# Autodesk Inventor assembly: Сборка2
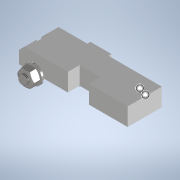
[picture p0: Inventor's stored thumbnail of the model, 180x180]
Saved by Autodesk Inventor 2022 (Build 260153000, 153)
## iProperties
Created: 2024-04-28
Part Number: Сборка2
Document SubType Name: Assembly
Designer: Pavel
Author: Pavel
## Documents named in this file (9)
- D:\BSUIR\КМЭКЭС\Сборка2.iam
- D:\BSUIR\КМЭКЭС\Исходники\Разрез\Деталь.ipt
- C:\Users\Pavel\Documents\Inventor\Content Center Files\R2022\ru-RU\Stud GOST 22032-76\Шпилька M10-6g×30 ГОСТ 22032-76.ipt
- C:\Users\Pavel\Documents\Inventor\Content Center Files\R2022\ru-RU\Washer 1 GOST 6402-78\Шайба 10Н ГОСТ 6402-78.ipt
- C:\Users\Pavel\Documents\Inventor\Content Center Files\R2022\ru-RU\GOST 5915-70\Гайка M10-6H ГОСТ 5915-70(1).ipt
- C:\Users\Pavel\Documents\Inventor\Content Center Files\R2022\ru-RU\Screw B GOST 17473-80\Винт B.M8-6gx25 ГОСТ 17473-80.ipt
- C:\Users\Pavel\Documents\Inventor\Content Center Files\R2022\ru-RU\Bolt GOST 7798-78\Болт M12-6g×60 ГОСТ 7798-70.ipt
- C:\Users\Pavel\Documents\Inventor\Content Center Files\R2022\ru-RU\GOST 11371-78  A\Шайба 12 ГОСТ 11371-78.ipt
- C:\Users\Pavel\Documents\Inventor\Content Center Files\R2022\ru-RU\GOST 5915-70\Гайка M12-6H ГОСТ 5915-70(1).ipt
## Components (8 placed, 8 different names)
1. Деталь:1 — Вставка:1, Вставка:2, Вставка:4, Вставка:5, Вставка:6
2. Шпилька ГОСТ 22032-76 M10-6g×30:1 — Вставка:1
3. Шайба 1 ГОСТ 6402-78 10Н:1 — Вставка:2, Вставка:3
4. Гайка ГОСТ 5915-70 M10:1 — Вставка:3
5. Винт B ГОСТ 17473-80 M8-6gx25:1 — Вставка:4
6. Болт ГОСТ 7798-70 M12-6g×60:1 — Вставка:5
7. Шайба  ГОСТ 11371-78 13:1 — Вставка:6, Вставка:7
8. Гайка ГОСТ 5915-70 M12:1 — Вставка:7
## Relationships (7: Insert 7)
- Вставка:1 [Insert] (-10 mm): Деталь:1 ↔ Шпилька ГОСТ 22032-76 M10-6g×30:1
- Вставка:2 [Insert]: Деталь:1 ↔ Шайба 1 ГОСТ 6402-78 10Н:1
- Вставка:3 [Insert]: Шайба 1 ГОСТ 6402-78 10Н:1 ↔ Гайка ГОСТ 5915-70 M10:1
- Вставка:4 [Insert]: Деталь:1 ↔ Винт B ГОСТ 17473-80 M8-6gx25:1
- Вставка:5 [Insert]: Деталь:1 ↔ Болт ГОСТ 7798-70 M12-6g×60:1
- Вставка:6 [Insert]: Деталь:1 ↔ Шайба  ГОСТ 11371-78 13:1
- Вставка:7 [Insert]: Шайба  ГОСТ 11371-78 13:1 ↔ Гайка ГОСТ 5915-70 M12:1
